# Autodesk Inventor assembly: Koła_tylne
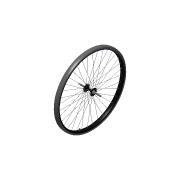
[picture p0: Inventor's stored thumbnail of the model, 180x180]
Saved by Autodesk Inventor 2015 (Build 190159000, 159)
## iProperties
Created: 2015-11-24
Part Number: Koła_tylne
Document SubType Name: Assembly
Designer: graaapsik
Author: graaapsik
## Documents named in this file (7)
- C:\Users\EriveltonDell\Documents\Centro Universitário da FEI\Wheelchair\CADEIRA DE RODAS - DESENHO\Model\Koło_tylne.iam
- C:\Users\EriveltonDell\Documents\Centro Universitário da FEI\Wheelchair\CADEIRA DE RODAS - DESENHO\Model\Opona_koła_tylnego.ipt
- C:\Users\EriveltonDell\Documents\Centro Universitário da FEI\Wheelchair\CADEIRA DE RODAS - DESENHO\Model\Obręcz_koła_tylnego.ipt
- C:\Users\EriveltonDell\Documents\Centro Universitário da FEI\Wheelchair\CADEIRA DE RODAS - DESENHO\Model\Piasta_koła_tylnego.iam
- Piasta.iam
- C:\Users\EriveltonDell\Documents\Centro Universitário da FEI\Wheelchair\CADEIRA DE RODAS - DESENHO\Model\Szprycha.iam
- C:\Users\EriveltonDell\Documents\Centro Universitário da FEI\Wheelchair\CADEIRA DE RODAS - DESENHO\Model\Dętka.iam
## Components (40 placed, 5 different names)
1. Piasta:1 [sub-assembly] — Kulkowe:2, Kąt:1, Kulkowe:3, Kąt:2, Obrotowe:3
2. Obręcz_koła_tylnego:1 — Zestawiający:1, Zestawiający:2, Równoległy:1, Walcowe:1, Równoległy:2, Obrotowe:1, Obrotowe:3
3. Dętka:1 [sub-assembly] — Równoległy:1, Walcowe:1, Obrotowe:1, Obrotowe:2
4. Opona_koła_tylnego:2 — Równoległy:2, Obrotowe:2
5. Szprycha:1 [sub-assembly] — Kulkowe:2, Zestawiający:1, Kąt:1
6. Szprycha:2 [sub-assembly]
7. Szprycha:3 [sub-assembly]
8. Szprycha:4 [sub-assembly]
9. Szprycha:5 [sub-assembly]
10. Szprycha:6 [sub-assembly]
11. Szprycha:7 [sub-assembly]
12. Szprycha:8 [sub-assembly]
13. Szprycha:9 [sub-assembly]
14. Szprycha:10 [sub-assembly]
15. Szprycha:11 [sub-assembly]
16. Szprycha:12 [sub-assembly]
17. Szprycha:13 [sub-assembly]
18. Szprycha:14 [sub-assembly]
19. Szprycha:15 [sub-assembly]
20. Szprycha:16 [sub-assembly]
21. Szprycha:17 [sub-assembly]
22. Szprycha:18 [sub-assembly]
23. Szprycha:19 [sub-assembly] — Zestawiający:2, Kulkowe:3, Kąt:2
24. Szprycha:20 [sub-assembly]
25. Szprycha:21 [sub-assembly]
26. Szprycha:22 [sub-assembly]
27. Szprycha:23 [sub-assembly]
28. Szprycha:24 [sub-assembly]
29. Szprycha:25 [sub-assembly]
30. Szprycha:26 [sub-assembly]
31. Szprycha:27 [sub-assembly]
32. Szprycha:28 [sub-assembly]
33. Szprycha:29 [sub-assembly]
34. Szprycha:30 [sub-assembly]
35. Szprycha:31 [sub-assembly]
36. Szprycha:32 [sub-assembly]
37. Szprycha:33 [sub-assembly]
38. Szprycha:34 [sub-assembly]
39. Szprycha:35 [sub-assembly]
40. Szprycha:36 [sub-assembly]
## Component patterns: Szyk szprych 1 (18 elements), Szyk szprych 2 (18 elements)
## Relationships (12: RevoluteJoint 3, BallJoint 2, Mate 2, Angle 2, Flush 2, CylindricalJoint 1)
- Kulkowe:2 [BallJoint]: Piasta:1 ↔ Szprycha:1
- Zestawiający:1 [Mate]: Obręcz_koła_tylnego:1 ↔ Szprycha:1
- Kąt:1 [Angle] (96.49 deg): Piasta:1 ↔ Szprycha:1
- Zestawiający:2 [Mate]: Obręcz_koła_tylnego:1 ↔ Szprycha:19
- Kulkowe:3 [BallJoint]: Piasta:1 ↔ Szprycha:19
- Kąt:2 [Angle] (95.94 deg): Piasta:1 ↔ Szprycha:19
- Równoległy:1 [Flush]: Obręcz_koła_tylnego:1 ↔ Dętka:1
- Walcowe:1 [CylindricalJoint]: Obręcz_koła_tylnego:1 ↔ Dętka:1
- Równoległy:2 [Flush]: Obręcz_koła_tylnego:1 ↔ Opona_koła_tylnego:2
- Obrotowe:1 [RevoluteJoint]: Obręcz_koła_tylnego:1 ↔ Dętka:1
- Obrotowe:2 [RevoluteJoint]: Dętka:1 ↔ Opona_koła_tylnego:2
- Obrotowe:3 [RevoluteJoint]: Piasta:1 ↔ Obręcz_koła_tylnego:1
